# Autodesk Inventor assembly: Gearbox Assembly_MIR
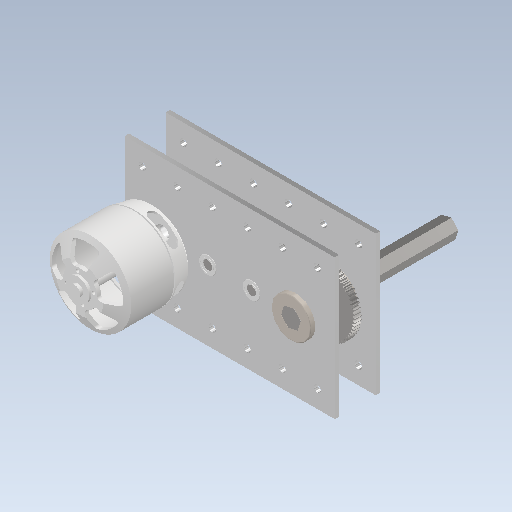
[picture p0: Inventor's stored thumbnail of the model, 512x512]
Saved by Autodesk Inventor 2023 (Build 270158000, 158)
## iProperties
Created: 2023-02-14
Part Number: Gearbox Assembly_MIR
Document SubType Name: Assembly
Designer: Dave
Mass: 682.162 g
Surface Area: 1267.39 cm^2
Volume: 183.282 cm^3
Density: 3.72192 g/cm^3
Author: Dave
## Documents named in this file (12)
- C:\Users\Dave\Documents\GitHub\BehrendURCMechanical\CAD\Chassis\GearBox\Final Gears and Assemblies\Gearbox Assembly_MIR.iam
- C:\Users\Dave\Documents\GitHub\BehrendURCMechanical\CAD\Chassis\GearBox\Final Gears and Assemblies\CH-1-01-20T_Drive Gear_MIR.ipt
- C:\Users\Dave\Documents\GitHub\BehrendURCMechanical\CAD\Chassis\GearBox\Final Gears and Assemblies\CH-1-01-60T_Output_MIR.ipt
- C:\Users\Dave\Documents\GitHub\BehrendURCMechanical\CAD\Chassis\GearBox\Final Gears and Assemblies\CH-1-01-20T_Idler_MIR.ipt
- C:\Users\Dave\Documents\GitHub\BehrendURCMechanical\CAD\Chassis\GearBox\Final Gears and Assemblies\CH-1-01-60T_Idler_MIR.ipt
- C:\Users\Dave\Documents\GitHub\BehrendURCMechanical\CAD\Chassis\GearBox\Housing\CH-1-02-RearGearboxHousingMotorSide_MIR.ipt
- C:\Users\Dave\Documents\GitHub\BehrendURCMechanical\CAD\Chassis\GearBox\Drive Motor Shaft Coupler_MIR.ipt
- C:\Users\Dave\Documents\GitHub\BehrendURCMechanical\CAD\Chassis\GearBox\Drive Motor_MIR.ipt
- C:\Users\Dave\Documents\GitHub\BehrendURCMechanical\CAD\Chassis\GearBox\Ch-1-01-0.5x4.5HexShaft_MIR.ipt
- C:\Users\Dave\Documents\GitHub\BehrendURCMechanical\CAD\Chassis\GearBox\CH-1-01-0.25x1.875SmoothShaft_MIR.ipt
- C:\Users\Dave\Documents\GitHub\BehrendURCMechanical\CAD\Chassis\GearBox\CH-1-01-0.5HexBearing_MIR.ipt
- C:\Users\Dave\Documents\GitHub\BehrendURCMechanical\CAD\Chassis\GearBox\CH-1-01-0.25IDSmoothBoreBearing_MIR.ipt
## Components (19 placed, 11 different names)
1. CH-1-01-20T_Drive Gear_MIR:1 — Insert:3
2. CH-1-01-60T_Output_MIR:1 — Mate:5, Mate:7, Mate:6
3. CH-1-01-20T_Idler_MIR:1 — Insert:1, Mate:2
4. CH-1-01-60T_Idler_MIR:1 — Mate:5, Insert:2, Mate:3
5. CH-1-01-20T_Idler_MIR:2 — Insert:2, Mate:4
6. CH-1-01-60T_Idler_MIR:2 — Mate:3, Insert:1, Mate:1
7. CH-1-02-RearGearboxHousingMotorSide_MIR:1 — Mate:4, Mate:2, Angle:1, Flush:2, Flush:1, Insert:5, Insert:10, Insert:6, Insert:7
8. CH-1-02-RearGearboxHousingMotorSide_MIR:2 — Mate:7, Mate:6, Flush:2, Flush:1, Insert:11, Insert:8, Insert:9
9. Drive Motor Shaft Coupler_MIR:1 — Insert:5, Mate:1, Insert:3, Insert:4
10. Drive Motor_MIR:1 — Insert:4
11. Ch-1-01-0.5x4.5HexShaft_MIR:1 — Mate:9, Mate:8, Flush:3
12. CH-1-01-0.25x1.875SmoothShaft_MIR:1 — Insert:13
13. CH-1-01-0.25x1.875SmoothShaft_MIR:2 — Insert:12
14. CH-1-01-0.5HexBearing_MIR:1 — Insert:11
15. CH-1-01-0.5HexBearing_MIR:2 — Mate:9, Mate:8, Flush:3, Insert:10
16. CH-1-01-0.25IDSmoothBoreBearing_MIR:1 — Insert:12, Insert:6
17. CH-1-01-0.25IDSmoothBoreBearing_MIR:2 — Insert:13, Insert:7
18. CH-1-01-0.25IDSmoothBoreBearing_MIR:3 — Insert:8
19. CH-1-01-0.25IDSmoothBoreBearing_MIR:4 — Insert:9
## Relationships (26: Insert 13, Mate 9, Flush 3, Angle 1)
- Mate:5: CH-1-01-60T_Output_MIR:1 ↔ CH-1-01-60T_Idler_MIR:1
- Insert:2: CH-1-01-60T_Idler_MIR:1 ↔ CH-1-01-20T_Idler_MIR:2
- Mate:3: CH-1-01-60T_Idler_MIR:1 ↔ CH-1-01-60T_Idler_MIR:2
- Insert:1: CH-1-01-20T_Idler_MIR:1 ↔ CH-1-01-60T_Idler_MIR:2
- Mate:4: CH-1-01-20T_Idler_MIR:2 ↔ CH-1-02-RearGearboxHousingMotorSide_MIR:1
- Mate:2: CH-1-01-20T_Idler_MIR:1 ↔ CH-1-02-RearGearboxHousingMotorSide_MIR:1
- Angle:1 (0 deg): CH-1-02-RearGearboxHousingMotorSide_MIR:1
- Mate:7 (1.5875 mm): CH-1-01-60T_Output_MIR:1 ↔ CH-1-02-RearGearboxHousingMotorSide_MIR:2
- Mate:6: CH-1-01-60T_Output_MIR:1 ↔ CH-1-02-RearGearboxHousingMotorSide_MIR:2
- Flush:2: CH-1-02-RearGearboxHousingMotorSide_MIR:1 ↔ CH-1-02-RearGearboxHousingMotorSide_MIR:2
- Flush:1: CH-1-02-RearGearboxHousingMotorSide_MIR:1 ↔ CH-1-02-RearGearboxHousingMotorSide_MIR:2
- Insert:5: CH-1-02-RearGearboxHousingMotorSide_MIR:1 ↔ Drive Motor Shaft Coupler_MIR:1
- Mate:1: CH-1-01-60T_Idler_MIR:2 ↔ Drive Motor Shaft Coupler_MIR:1
- Insert:3: CH-1-01-20T_Drive Gear_MIR:1 ↔ Drive Motor Shaft Coupler_MIR:1
- Insert:4: Drive Motor Shaft Coupler_MIR:1 ↔ Drive Motor_MIR:1
- Insert:11: CH-1-02-RearGearboxHousingMotorSide_MIR:2 ↔ CH-1-01-0.5HexBearing_MIR:1
- Mate:9: Ch-1-01-0.5x4.5HexShaft_MIR:1 ↔ CH-1-01-0.5HexBearing_MIR:2
- Mate:8: Ch-1-01-0.5x4.5HexShaft_MIR:1 ↔ CH-1-01-0.5HexBearing_MIR:2
- Flush:3: Ch-1-01-0.5x4.5HexShaft_MIR:1 ↔ CH-1-01-0.5HexBearing_MIR:2
- Insert:10: CH-1-02-RearGearboxHousingMotorSide_MIR:1 ↔ CH-1-01-0.5HexBearing_MIR:2
- Insert:12: CH-1-01-0.25x1.875SmoothShaft_MIR:2 ↔ CH-1-01-0.25IDSmoothBoreBearing_MIR:1
- Insert:6: CH-1-02-RearGearboxHousingMotorSide_MIR:1 ↔ CH-1-01-0.25IDSmoothBoreBearing_MIR:1
- Insert:13: CH-1-01-0.25x1.875SmoothShaft_MIR:1 ↔ CH-1-01-0.25IDSmoothBoreBearing_MIR:2
- Insert:7: CH-1-02-RearGearboxHousingMotorSide_MIR:1 ↔ CH-1-01-0.25IDSmoothBoreBearing_MIR:2
- Insert:8: CH-1-02-RearGearboxHousingMotorSide_MIR:2 ↔ CH-1-01-0.25IDSmoothBoreBearing_MIR:3
- Insert:9: CH-1-02-RearGearboxHousingMotorSide_MIR:2 ↔ CH-1-01-0.25IDSmoothBoreBearing_MIR:4
